# Autodesk Inventor assembly: IntakeSlides2.0
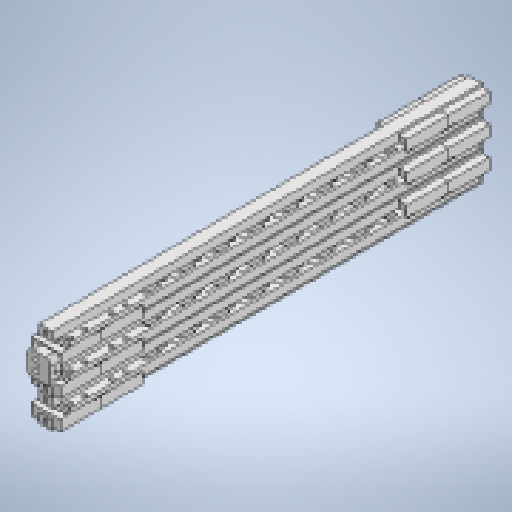
[picture p0: Inventor's stored thumbnail of the model, 512x512]
Saved by Autodesk Inventor 2023 (Build 270158000, 158)
## iProperties
Created: 2022-09-16
Part Number: IntakeSlides2.0
Document SubType Name: Assembly
Designer: deli
Author: deli
## Documents named in this file (3)
- C:\Users\deli\OneDrive - Eastside Preparatory School\FTC\8103-power-play\CAD\IntakeSlides2.0.iam
- C:\Users\deli\OneDrive - Eastside Preparatory School\FTC\8103-power-play\CAD\steelSlides.iam
- C:\Users\deli\OneDrive - Eastside Preparatory School\FTC\8103-power-play\CAD\SlideStopBearingHolder.ipt
## Components (7 placed, 2 different names)
1. steelSlides:1 [sub-assembly] — Mate:1, Flush:1, Flush:2, Mate:8, Mate:14
2. steelSlides:2 [sub-assembly] — Mate:1, Flush:1, Flush:2, Mate:2, Flush:3, Flush:4, Mate:5, Mate:6, Mate:7, Mate:11, Mate:12, Mate:13
3. steelSlides:3 [sub-assembly] — Mate:2, Flush:3, Flush:4, Mate:3, Mate:4, Mate:9, Mate:10
4. SlideStopBearingHolder:1 — Mate:3, Mate:4, Mate:5
5. SlideStopBearingHolder:2 — Mate:6, Mate:7, Mate:8
6. SlideStopBearingHolder:3 — Mate:9, Mate:10, Mate:11
7. SlideStopBearingHolder:4 — Mate:12, Mate:13, Mate:14
## Relationships (18: Mate 14, Flush 4)
- Mate:1: steelSlides:1 ↔ steelSlides:2
- Flush:1: steelSlides:1 ↔ steelSlides:2
- Flush:2: steelSlides:1 ↔ steelSlides:2
- Mate:2: steelSlides:2 ↔ steelSlides:3
- Flush:3: steelSlides:2 ↔ steelSlides:3
- Flush:4: steelSlides:2 ↔ steelSlides:3
- Mate:3: steelSlides:3 ↔ SlideStopBearingHolder:1
- Mate:4: steelSlides:3 ↔ SlideStopBearingHolder:1
- Mate:5: steelSlides:2 ↔ SlideStopBearingHolder:1
- Mate:6: steelSlides:2 ↔ SlideStopBearingHolder:2
- Mate:7: steelSlides:2 ↔ SlideStopBearingHolder:2
- Mate:8: steelSlides:1 ↔ SlideStopBearingHolder:2
- Mate:9: steelSlides:3 ↔ SlideStopBearingHolder:3
- Mate:10: steelSlides:3 ↔ SlideStopBearingHolder:3
- Mate:11: steelSlides:2 ↔ SlideStopBearingHolder:3
- Mate:12: steelSlides:2 ↔ SlideStopBearingHolder:4
- Mate:13: steelSlides:2 ↔ SlideStopBearingHolder:4
- Mate:14: steelSlides:1 ↔ SlideStopBearingHolder:4
